# Autodesk Inventor assembly: Selection_Ramp 1
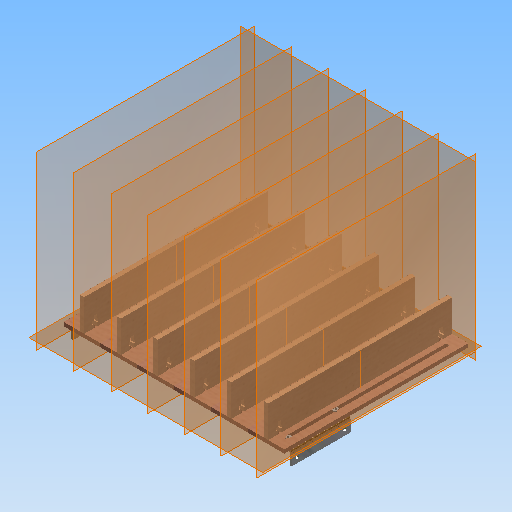
[picture p0: Inventor's stored thumbnail of the model, 512x512]
Saved by Autodesk Inventor 2018.1 (Build 221171000, 171)
## iProperties
Created: 2019-02-07
Part Number: Selection_Ramp 1
Document SubType Name: Assembly
Designer: James
Author: James
## Documents named in this file (6)
- C:\Users\admin\Desktop\Ball-Machine\Prototype CAD\Selection Sort - 40mm\Prototype_Ramp Long.iam
- C:\Users\admin\Desktop\Ball-Machine\Prototype CAD\Selection Sort - 40mm\Nyloc Nut - M4.ipt
- C:\Users\admin\Desktop\Ball-Machine\Prototype CAD\Selection Sort - 40mm\Prototype_Angle Bracket 1.ipt
- C:\Users\admin\Desktop\Ball-Machine\Prototype CAD\Selection Sort - 40mm\Socket Csk Screw - (A2) - M4 x  12.ipt
- C:\Users\admin\Desktop\Ball-Machine\Prototype CAD\Selection Sort - 40mm\Prototype_Ramp Long.ipt
- C:\Users\admin\Desktop\Ball-Machine\Prototype CAD\Selection Sort - 40mm\Prototype_Ramp Long Piece.ipt
## Components (17 placed, 5 different names)
1. Prototype_Ramp Long:1 — Flush:1, Flush:2, Flush:3, Mate:22, Flush:10, Mate:23, Mate:24, Mate:25, Mate:26, Tangent:3, Tangent:4, Tangent:5, Tangent:6, Mate:35, Mate:36, Mate:37, Flush:11, Mate:38, Mate:39, Mate:40, Flush:12, Flush:13
2. Nyloc Nut - M4:25 — Mate:27, Mate:30
3. Prototype_Angle Bracket 1:1 — Mate:22, Flush:10, Mate:23, Mate:24, Mate:27, Mate:28
4. Socket Csk Screw - (A2) - M4 x  12:2 — Mate:25, Tangent:4, Mate:30
5. Nyloc Nut - M4:26 — Mate:28, Mate:29
6. Socket Csk Screw - (A2) - M4 x  12:1 — Mate:26, Tangent:3, Mate:29
7. Nyloc Nut - M4:27
8. Prototype_Angle Bracket 1:2 — Mate:37, Flush:11, Mate:38, Mate:39
9. Socket Csk Screw - (A2) - M4 x  12:3 — Tangent:6, Mate:35
10. Nyloc Nut - M4:28
11. Socket Csk Screw - (A2) - M4 x  12:4 — Tangent:5, Mate:36
12. Prototype_Ramp Long Piece:1 — Mate:40, Flush:12, Flush:13
13. Prototype_Ramp Long Piece:2
14. Prototype_Ramp Long Piece:3
15. Prototype_Ramp Long Piece:4
16. Prototype_Ramp Long Piece:5
17. Prototype_Ramp Long Piece:6
## Component patterns: (6 elements, first: Prototype_Ramp Long Piece:1)
## Relationships (30: Mate 19, Flush 7, Tangent 4)
- Flush:1: Prototype_Ramp Long:1
- Flush:2: Prototype_Ramp Long:1
- Flush:3: Prototype_Ramp Long:1
- Mate:22: Prototype_Ramp Long:1 ↔ Prototype_Angle Bracket 1:1
- Flush:10: Prototype_Ramp Long:1 ↔ Prototype_Angle Bracket 1:1
- Mate:23: Prototype_Ramp Long:1 ↔ Prototype_Angle Bracket 1:1
- Mate:24: Prototype_Ramp Long:1 ↔ Prototype_Angle Bracket 1:1
- Mate:25: Prototype_Ramp Long:1 ↔ Socket Csk Screw - (A2) - M4 x  12:2
- Mate:26: Prototype_Ramp Long:1 ↔ Socket Csk Screw - (A2) - M4 x  12:1
- Mate:27: Nyloc Nut - M4:25 ↔ Prototype_Angle Bracket 1:1
- Mate:28: Prototype_Angle Bracket 1:1 ↔ Nyloc Nut - M4:26
- Tangent:3: Prototype_Ramp Long:1 ↔ Socket Csk Screw - (A2) - M4 x  12:1
- Tangent:4: Prototype_Ramp Long:1 ↔ Socket Csk Screw - (A2) - M4 x  12:2
- Mate:29: Nyloc Nut - M4:26 ↔ Socket Csk Screw - (A2) - M4 x  12:1
- Mate:30: Nyloc Nut - M4:25 ↔ Socket Csk Screw - (A2) - M4 x  12:2
- [Mate]: Nyloc Nut - M4:27 ↔ Prototype_Angle Bracket 1:2
- [Mate]: Prototype_Angle Bracket 1:2 ↔ Nyloc Nut - M4:28
- [Mate]: Nyloc Nut - M4:28 ↔ Socket Csk Screw - (A2) - M4 x  12:4
- [Mate]: Nyloc Nut - M4:27 ↔ Socket Csk Screw - (A2) - M4 x  12:3
- Tangent:5: Prototype_Ramp Long:1 ↔ Socket Csk Screw - (A2) - M4 x  12:4
- Tangent:6: Prototype_Ramp Long:1 ↔ Socket Csk Screw - (A2) - M4 x  12:3
- Mate:35: Prototype_Ramp Long:1 ↔ Socket Csk Screw - (A2) - M4 x  12:3
- Mate:36: Prototype_Ramp Long:1 ↔ Socket Csk Screw - (A2) - M4 x  12:4
- Mate:37: Prototype_Ramp Long:1 ↔ Prototype_Angle Bracket 1:2
- Flush:11: Prototype_Ramp Long:1 ↔ Prototype_Angle Bracket 1:2
- Mate:38: Prototype_Ramp Long:1 ↔ Prototype_Angle Bracket 1:2
- Mate:39: Prototype_Ramp Long:1 ↔ Prototype_Angle Bracket 1:2
- Mate:40: Prototype_Ramp Long:1 ↔ Prototype_Ramp Long Piece:1
- Flush:12 (22 mm): Prototype_Ramp Long:1 ↔ Prototype_Ramp Long Piece:1
- Flush:13: Prototype_Ramp Long:1 ↔ Prototype_Ramp Long Piece:1
## Named parameters: d52_d46 = 0 mm, d53_d47 = 0 mm, d54_d50 = 0 mm, d55_d51 = 0 mm
